# Autodesk Inventor assembly: LowerBackLink
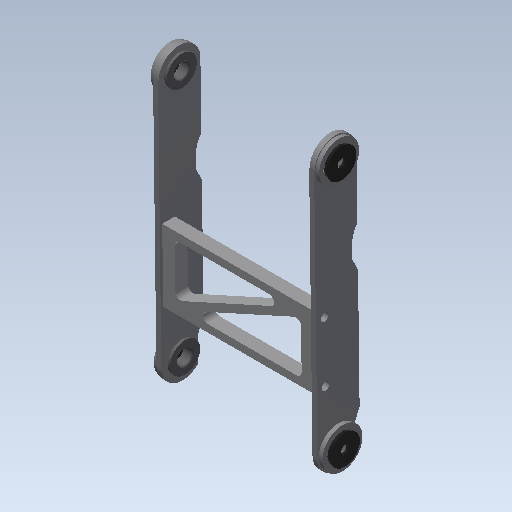
[picture p0: Inventor's stored thumbnail of the model, 512x512]
Saved by Autodesk Inventor 2020.4 (Build 244396000, 396)
## iProperties
Created: 2016-08-23
Part Number: LowerBackLink
Material: 一般
Document SubType Name: Assembly
Designer: hiro
Mass: 27.0677 g
Surface Area: 148.123 cm^2
Volume: 12.1706 cm^3
Density: 2.22402 g/cm^3
Author: hiro
## Documents named in this file (6)
- C:\Users\Masato\Documents\Inventor\CIT Brains_Inventor\OpenPlatform_ver3_0\下半身\リンク\LowerBackLink.iam
- C:\Users\Masato\Documents\Inventor\CIT Brains_Inventor\OpenPlatform_ver3_0\下半身\リンク\リンク_メインフレーム_6_1.ipt
- C:\Users\Masato\Documents\Inventor\CIT Brains_Inventor\OpenPlatform_ver3_0\下半身\リンク\リンク_ふくらはぎ_サブフレーム_1_2.ipt
- C:\Users\Masato\Documents\Inventor\CIT Brains_Inventor\OpenPlatform_ver3_0\Ready_Made\UUW-0312-10BH.ipt
- C:\Users\Masato\Documents\Inventor\CIT Brains_Inventor\OpenPlatform_ver3_0\Ready_Made\LFW-0815.ipt
- C:\Users\Masato\Documents\Inventor\CIT Brains_Inventor\OpenPlatform_ver3_0\Ready_Made\80F-0603.ipt
## Components (15 placed, 5 different names)
1. リンク_メインフレーム_6_1:1 — 挿入:17, 挿入:21, 挿入:22, 挿入:27, 挿入:28, 挿入:31
2. リンク_メインフレーム_6_1:2 — 挿入:18, 挿入:23, 挿入:24, 挿入:25, 挿入:26, 挿入:32
3. UUW-0312-10BH:1 — 挿入:30
4. UUW-0312-10BH:2 — 挿入:29
5. UUW-0312-10BH:3 — 挿入:20
6. UUW-0312-10BH:4 — 挿入:19
7. LFW-0815:1 — 挿入:18, 挿入:20
8. LFW-0815:2 — 挿入:17, 挿入:19
9. リンク_ふくらはぎ_サブフレーム_1_2:1 — 挿入:21, 挿入:22, 挿入:23, 挿入:24
10. 80F-0603:1 — 挿入:28
11. 80F-0603:2 — 挿入:27
12. 80F-0603:3 — 挿入:26
13. 80F-0603:4 — 挿入:25
14. LFW-0815:3 — 挿入:29, 挿入:32
15. LFW-0815:4 — 挿入:30, 挿入:31
## Relationships (16: Insert 16)
- 挿入:17 [Insert]: リンク_メインフレーム_6_1:1 ↔ LFW-0815:2
- 挿入:18 [Insert]: リンク_メインフレーム_6_1:2 ↔ LFW-0815:1
- 挿入:19 [Insert]: UUW-0312-10BH:4 ↔ LFW-0815:2
- 挿入:20 [Insert]: UUW-0312-10BH:3 ↔ LFW-0815:1
- 挿入:21 [Insert]: リンク_メインフレーム_6_1:1 ↔ リンク_ふくらはぎ_サブフレーム_1_2:1
- 挿入:22 [Insert]: リンク_メインフレーム_6_1:1 ↔ リンク_ふくらはぎ_サブフレーム_1_2:1
- 挿入:23 [Insert]: リンク_メインフレーム_6_1:2 ↔ リンク_ふくらはぎ_サブフレーム_1_2:1
- 挿入:24 [Insert]: リンク_メインフレーム_6_1:2 ↔ リンク_ふくらはぎ_サブフレーム_1_2:1
- 挿入:25 [Insert]: リンク_メインフレーム_6_1:2 ↔ 80F-0603:4
- 挿入:26 [Insert]: リンク_メインフレーム_6_1:2 ↔ 80F-0603:3
- 挿入:27 [Insert]: リンク_メインフレーム_6_1:1 ↔ 80F-0603:2
- 挿入:28 [Insert]: リンク_メインフレーム_6_1:1 ↔ 80F-0603:1
- 挿入:29 [Insert]: UUW-0312-10BH:2 ↔ LFW-0815:3
- 挿入:30 [Insert]: UUW-0312-10BH:1 ↔ LFW-0815:4
- 挿入:31 [Insert]: リンク_メインフレーム_6_1:1 ↔ LFW-0815:4
- 挿入:32 [Insert]: リンク_メインフレーム_6_1:2 ↔ LFW-0815:3
